# Autodesk Inventor assembly: Mold Design1
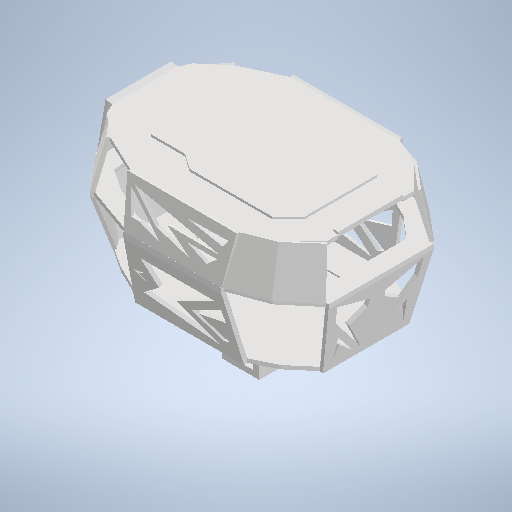
[picture p0: Inventor's stored thumbnail of the model, 512x512]
Saved by Autodesk Inventor 2025.2 (Build 292293000, 293)
## iProperties
Created: 2025-04-15
Part Number: Mold Design1
Document SubType Name: Assembly
Designer: ziyuz
Author: ziyuz
## Documents named in this file (6)
- F:\autoeskinvetersave\lanche\Mold Design1.iam
- F:\autoeskinvetersave\lanche\Part1EDDV4.ipt
- F:\autoeskinvetersave\lanche\Part2EDD.ipt
- F:\autoeskinvetersave\lanche\Part3EDD.ipt
- F:\autoeskinvetersave\lanche\Part4EDD.ipt
- F:\autoeskinvetersave\lanche\Part6.ipt
## Components (6 placed, 5 different names)
1. Part1EDDV4:1 — Rigid:1, Rotational:1, Rotational:2, Rotational:3, Mate:1, Mate:2, Mate:3
2. Part2EDD:1 — Rigid:1
3. Part3EDD:1 — Rotational:2
4. Part3EDD:2 — Rotational:3
5. Part4EDD:1 — Rotational:1
6. Part6:1 — Mate:1, Mate:2, Mate:3
## Relationships (7: RevoluteJoint 3, Mate 3, WeldJoint 1)
- Rigid:1 [WeldJoint] (12.5 mm): Part1EDDV4:1 ↔ Part2EDD:1
- Rotational:1 [RevoluteJoint] (-0.5 mm): Part1EDDV4:1 ↔ Part4EDD:1
- Rotational:2 [RevoluteJoint]: Part1EDDV4:1 ↔ Part3EDD:1
- Rotational:3 [RevoluteJoint]: Part1EDDV4:1 ↔ Part3EDD:2
- Mate:1: Part1EDDV4:1 ↔ Part6:1
- Mate:2: Part1EDDV4:1 ↔ Part6:1
- Mate:3: Part1EDDV4:1 ↔ Part6:1
